# Autodesk Inventor assembly: FakeMachineV2
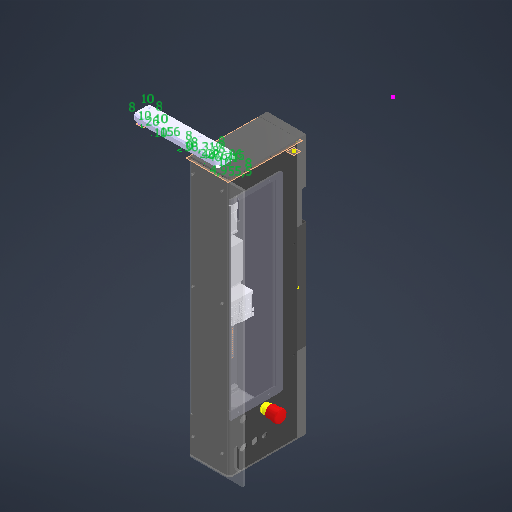
[picture p0: Inventor's stored thumbnail of the model, 512x512]
Saved by Autodesk Inventor 2026.1 (Build 301233020, 233B)
## iProperties
Created: 2025-04-28
Part Number: FakeMachineV2
Document SubType Name: Assembly
Designer: iopeter
Author: iopeter
## Documents named in this file (19)
- C:\Users\neume\Desktop\MCI\Robotik_Projekt\Optimierung-Laboraufgabe-Robotik\Abgabe_Optimierung_Robotik\Konstruktion\Inventor_ConveyorTracking\FakeMachineV2.iam
- C:\Users\neume\Desktop\MCI\Robotik_Projekt\Optimierung-Laboraufgabe-Robotik\Abgabe_Optimierung_Robotik\Konstruktion\Inventor_ConveyorTracking\u-blech-fakemachine.ipt
- C:\Users\neume\Desktop\MCI\Robotik_Projekt\Optimierung-Laboraufgabe-Robotik\Abgabe_Optimierung_Robotik\Konstruktion\Inventor_ConveyorTracking\Elektro_V2.ipt
- C:\Users\neume\Desktop\MCI\Robotik_Projekt\Optimierung-Laboraufgabe-Robotik\Abgabe_Optimierung_Robotik\Konstruktion\Inventor_ConveyorTracking\Werkstückträger.ipt
- C:\Users\neume\Desktop\MCI\Robotik_Projekt\Optimierung-Laboraufgabe-Robotik\Abgabe_Optimierung_Robotik\Konstruktion\Inventor_ConveyorTracking\Rampe_V2.ipt
- C:\Users\neume\Desktop\MCI\Robotik_Projekt\Optimierung-Laboraufgabe-Robotik\Abgabe_Optimierung_Robotik\Konstruktion\Inventor_ConveyorTracking\Endstueck_Harting.ipt
- C:\Users\neume\Desktop\MCI\Robotik_Projekt\Optimierung-Laboraufgabe-Robotik\Abgabe_Optimierung_Robotik\Konstruktion\Inventor_ConveyorTracking\983-002-ZR-40-80-585-10-K.ipt
- C:\Users\neume\Desktop\MCI\Robotik_Projekt\Optimierung-Laboraufgabe-Robotik\Abgabe_Optimierung_Robotik\Konstruktion\Inventor_ConveyorTracking\Trennblech_v1.ipt
- C:\Users\neume\Desktop\MCI\Robotik_Projekt\Optimierung-Laboraufgabe-Robotik\Abgabe_Optimierung_Robotik\Konstruktion\Inventor_ConveyorTracking\Plexi_Teileband.ipt
- C:\Users\neume\Desktop\MCI\Robotik_Projekt\Optimierung-Laboraufgabe-Robotik\Abgabe_Optimierung_Robotik\Konstruktion\Inventor_ConveyorTracking\halter_induktivsensor_klein.ipt
- C:\Users\neume\Desktop\MCI\Robotik_Projekt\Optimierung-Laboraufgabe-Robotik\Abgabe_Optimierung_Robotik\Konstruktion\Inventor_ConveyorTracking\Comus PGN-SP-002 v1.ipt
- C:\Users\neume\Desktop\MCI\Robotik_Projekt\Optimierung-Laboraufgabe-Robotik\Abgabe_Optimierung_Robotik\Konstruktion\Inventor_ConveyorTracking\dc11_0001_001.ipt
- C:\Users\neume\Desktop\MCI\Robotik_Projekt\Optimierung-Laboraufgabe-Robotik\Abgabe_Optimierung_Robotik\Konstruktion\Inventor_ConveyorTracking\Endstueck_noHarting.ipt
- C:\Users\neume\Desktop\MCI\Robotik_Projekt\Optimierung-Laboraufgabe-Robotik\Abgabe_Optimierung_Robotik\Konstruktion\Inventor_ConveyorTracking\FakeMachine_Abdeckung.ipt
- C:\Users\neume\Desktop\MCI\Robotik_Projekt\Optimierung-Laboraufgabe-Robotik\Abgabe_Optimierung_Robotik\Konstruktion\Inventor_ConveyorTracking\LED_Dummy.ipt
- C:\Users\neume\Desktop\MCI\Robotik_Projekt\Optimierung-Laboraufgabe-Robotik\Abgabe_Optimierung_Robotik\Konstruktion\Inventor_ConveyorTracking\Plexiglasabdeckung.ipt
- C:\Users\neume\Desktop\MCI\Robotik_Projekt\Optimierung-Laboraufgabe-Robotik\Abgabe_Optimierung_Robotik\Konstruktion\Inventor_ConveyorTracking\seitliche_Abdeckung_Kabel.ipt
- C:\Users\neume\Desktop\MCI\Robotik_Projekt\Optimierung-Laboraufgabe-Robotik\Abgabe_Optimierung_Robotik\Konstruktion\Inventor_ConveyorTracking\item_0069153_notaus-_nothalt-taster_22m.ipt
- C:\Users\neume\Desktop\MCI\Robotik_Projekt\Optimierung-Laboraufgabe-Robotik\Abgabe_Optimierung_Robotik\Konstruktion\Inventor_ConveyorTracking\FakeMachine_Abdeckung_Mitte.ipt
## Components (28 placed, 18 different names)
1. u-blech-fakemachine:1 — Fluchtend:2, Fluchtend:3, Fluchtend:5, Fluchtend:6, Fluchtend:7, Fluchtend:9, Fluchtend:10, Fluchtend:11, Fluchtend:12, Fluchtend:15, Zylindrisch:1, Passend:38, Passend:40, Einfügen:3
2. Elektro_V2:1
3. Rampe_V2:1 — Fluchtend:2, Fluchtend:3, Passend:2, Passend:28, Passend:29, Passend:30
4. Endstueck_Harting:1 — Fluchtend:5, Passend:32
5. 983-002-ZR-40-80-585-10-K:1 — Fluchtend:6, Fluchtend:7, Passend:2, Passend:4, Passend:5, Passend:6, Passend:7, Passend:8, Passend:9, Passend:10, Passend:11, Passend:12, Passend:13, Passend:14, Passend:15, Passend:16, Passend:17, Passend:18, Passend:19, Passend:20, Passend:21, Passend:22, Passend:23, Fluchtend:8, Fluchtend:16, Passend:24, Passend:25
6. Werkstückträger:12 — Passend:22, Passend:23
7. Trennblech_v2:1 — Fluchtend:8, Fluchtend:9, Fluchtend:10, Fluchtend:11, Fluchtend:12, Passend:33, Passend:34
8. Plexi_Teileband:1 — Fluchtend:15, Planar:1, Passend:41
9. halter_induktivsensor_klein:1 — Fluchtend:16, Passend:26, Passend:27
10. Werkstückträger:13 — Passend:24, Passend:25
11. Comus PGN-SP-002 v1:1 — Passend:26, Passend:27
12. dc11_0001_001:1 — Passend:28, Passend:29, Passend:30
13. Endstueck_noHarting:1 — Passend:32, Einfügen:4
14. FakeMachine_Abdeckung:1 — Passend:33, Passend:34, Passend:36, Fluchtend:17, Fluchtend:18, Passend:39
15. LED_Dummy:1 — Passend:36
16. Plexiglasabdeckung:1 — Planar:1, Zylindrisch:1, Passend:40, Passend:41, Einfügen:3
17. seitliche_Abdeckung_Kabel:1 — Einfügen:4
18. item_0069153_notaus-_nothalt-taster_22m:1 — Passend:38
19. FakeMachine_Abdeckung_Mitte:1 — Fluchtend:17, Fluchtend:18, Passend:39
20. Werkstückträger:11 — Passend:20, Passend:21
21. Werkstückträger:10 — Passend:18, Passend:19
22. Werkstückträger:4 — Passend:4, Passend:5
23. Werkstückträger:7 — Passend:14, Passend:15
24. Werkstückträger:8 — Passend:16, Passend:17
25. Werkstückträger:9 — Passend:12, Passend:13
26. Werkstückträger:3 — Passend:10, Passend:11
27. Werkstückträger:2 — Passend:6, Passend:7
28. Werkstückträger:1 — Passend:8, Passend:9
## Relationships (54: Mate 36, Flush 14, Insert 2, PlanarJoint 1, CylindricalJoint 1)
- Fluchtend:2 [Flush]: u-blech-fakemachine:1 ↔ Rampe_V2:1
- Fluchtend:3 [Flush]: u-blech-fakemachine:1 ↔ Rampe_V2:1
- Fluchtend:5 [Flush]: u-blech-fakemachine:1 ↔ Endstueck_Harting:1
- Fluchtend:6 [Flush]: u-blech-fakemachine:1 ↔ 983-002-ZR-40-80-585-10-K:1
- Fluchtend:7 [Flush]: u-blech-fakemachine:1 ↔ 983-002-ZR-40-80-585-10-K:1
- Passend:2 [Mate] (85 mm): Rampe_V2:1 ↔ 983-002-ZR-40-80-585-10-K:1
- Passend:4 [Mate]: 983-002-ZR-40-80-585-10-K:1 ↔ Werkstückträger:4
- Passend:5 [Mate]: 983-002-ZR-40-80-585-10-K:1 ↔ Werkstückträger:4
- Passend:6 [Mate]: 983-002-ZR-40-80-585-10-K:1 ↔ Werkstückträger:2
- Passend:7 [Mate]: 983-002-ZR-40-80-585-10-K:1 ↔ Werkstückträger:2
- Passend:8 [Mate]: 983-002-ZR-40-80-585-10-K:1 ↔ Werkstückträger:1
- Passend:9 [Mate]: 983-002-ZR-40-80-585-10-K:1 ↔ Werkstückträger:1
- Passend:10 [Mate]: 983-002-ZR-40-80-585-10-K:1 ↔ Werkstückträger:3
- Passend:11 [Mate]: 983-002-ZR-40-80-585-10-K:1 ↔ Werkstückträger:3
- Passend:12 [Mate]: 983-002-ZR-40-80-585-10-K:1 ↔ Werkstückträger:9
- Passend:13 [Mate]: 983-002-ZR-40-80-585-10-K:1 ↔ Werkstückträger:9
- Passend:14 [Mate]: 983-002-ZR-40-80-585-10-K:1 ↔ Werkstückträger:7
- Passend:15 [Mate]: 983-002-ZR-40-80-585-10-K:1 ↔ Werkstückträger:7
- Passend:16 [Mate]: 983-002-ZR-40-80-585-10-K:1 ↔ Werkstückträger:8
- Passend:17 [Mate]: 983-002-ZR-40-80-585-10-K:1 ↔ Werkstückträger:8
- Passend:18 [Mate]: 983-002-ZR-40-80-585-10-K:1 ↔ Werkstückträger:10
- Passend:19 [Mate]: 983-002-ZR-40-80-585-10-K:1 ↔ Werkstückträger:10
- Passend:20 [Mate]: 983-002-ZR-40-80-585-10-K:1 ↔ Werkstückträger:11
- Passend:21 [Mate]: 983-002-ZR-40-80-585-10-K:1 ↔ Werkstückträger:11
- Passend:22 [Mate]: 983-002-ZR-40-80-585-10-K:1 ↔ Werkstückträger:12
- Passend:23 [Mate]: 983-002-ZR-40-80-585-10-K:1 ↔ Werkstückträger:12
- Fluchtend:8 [Flush]: 983-002-ZR-40-80-585-10-K:1 ↔ Trennblech_v2:1
- Fluchtend:9 [Flush]: u-blech-fakemachine:1 ↔ Trennblech_v2:1
- Fluchtend:10 [Flush]: u-blech-fakemachine:1 ↔ Trennblech_v2:1
- Fluchtend:11 [Flush]: u-blech-fakemachine:1 ↔ Trennblech_v2:1
- Fluchtend:12 [Flush]: u-blech-fakemachine:1 ↔ Trennblech_v2:1
- Fluchtend:15 [Flush] (3 mm): u-blech-fakemachine:1 ↔ Plexi_Teileband:1
- Fluchtend:16 [Flush]: 983-002-ZR-40-80-585-10-K:1 ↔ halter_induktivsensor_klein:1
- Passend:24 [Mate]: 983-002-ZR-40-80-585-10-K:1 ↔ Werkstückträger:13
- Passend:25 [Mate]: 983-002-ZR-40-80-585-10-K:1 ↔ Werkstückträger:13
- Passend:26 [Mate]: halter_induktivsensor_klein:1 ↔ Comus PGN-SP-002 v1:1
- Passend:27 [Mate]: halter_induktivsensor_klein:1 ↔ Comus PGN-SP-002 v1:1
- Passend:28 [Mate]: Rampe_V2:1 ↔ dc11_0001_001:1
- Passend:29 [Mate]: Rampe_V2:1 ↔ dc11_0001_001:1
- Passend:30 [Mate]: Rampe_V2:1 ↔ dc11_0001_001:1
- Passend:32 [Mate]: Endstueck_Harting:1 ↔ Endstueck_noHarting:1
- Passend:33 [Mate]: Trennblech_v2:1 ↔ FakeMachine_Abdeckung:1
- Passend:34 [Mate]: Trennblech_v2:1 ↔ FakeMachine_Abdeckung:1
- Passend:36 [Mate]: FakeMachine_Abdeckung:1 ↔ LED_Dummy:1
- Planar:1: Plexi_Teileband:1 ↔ Plexiglasabdeckung:1
- Zylindrisch:1 [CylindricalJoint]: u-blech-fakemachine:1 ↔ Plexiglasabdeckung:1
- Passend:38 [Mate]: u-blech-fakemachine:1 ↔ item_0069153_notaus-_nothalt-taster_22m:1
- Fluchtend:17 [Flush]: FakeMachine_Abdeckung:1 ↔ FakeMachine_Abdeckung_Mitte:1
- Fluchtend:18 [Flush]: FakeMachine_Abdeckung:1 ↔ FakeMachine_Abdeckung_Mitte:1
- Passend:39 [Mate]: FakeMachine_Abdeckung:1 ↔ FakeMachine_Abdeckung_Mitte:1
- Passend:40 [Mate]: u-blech-fakemachine:1 ↔ Plexiglasabdeckung:1
- Passend:41 [Mate]: Plexi_Teileband:1 ↔ Plexiglasabdeckung:1
- Einfügen:3 [Insert]: u-blech-fakemachine:1 ↔ Plexiglasabdeckung:1
- Einfügen:4 [Insert]: Endstueck_noHarting:1 ↔ seitliche_Abdeckung_Kabel:1
